# Autodesk Inventor assembly: centerArm
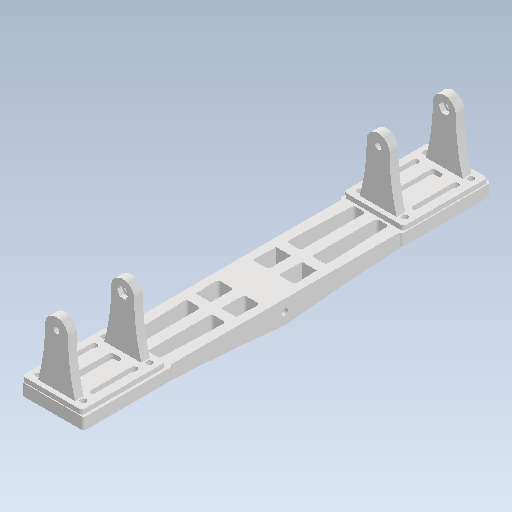
[picture p0: Inventor's stored thumbnail of the model, 512x512]
Saved by Autodesk Inventor 2020 (Build 240168000, 168)
## iProperties
Created: 2019-07-15
Part Number: centerArm
Document SubType Name: Assembly
Designer: Sean
Author: Sean
## Documents named in this file (4)
- C:\Users\Sean\Documents\Inventor\BalanceStand\centerArm.iam
- C:\Users\Sean\Documents\Inventor\BalanceStand\centerArm.ipt
- C:\Users\Sean\Documents\Inventor\BalanceStand\sideArmsHolder.ipt
- C:\Users\Sean\Documents\Inventor\BalanceStand\sideArmsHolder_MIR.ipt
## Components (3 placed, 3 different names)
1. centerArm:1 — Flush:1, Flush:2, Mate:1
2. sideArmsHolder:1 — Flush:1, Flush:2, Mate:1
3. sideArmsHolder_MIR:1
## Relationships (3: Flush 2, Mate 1)
- Flush:1 (99.06 mm): centerArm:1 ↔ sideArmsHolder:1
- Flush:2 (1.2319 mm): centerArm:1 ↔ sideArmsHolder:1
- Mate:1: centerArm:1 ↔ sideArmsHolder:1
